# Autodesk Inventor assembly: DriveTrainPlate
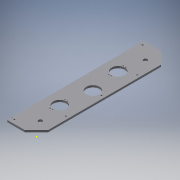
[picture p0: Inventor's stored thumbnail of the model, 180x180]
Saved by Autodesk Inventor 2017 (Build 210142000, 142)
## iProperties
Created: 2016-09-21
Part Number: DriveTrainPlate
Document SubType Name: Assembly
Designer: RoboticsUser
Author: RoboticsUser
## Documents named in this file (3)
- C:\Robotics\CAD\2016-17_CAD\DrainTrainPlate2.0.iam
- C:\Robotics\CAD\2016-17_CAD\DriveTrainPlate.ipt
- C:\Robotics\CAD\2016-17_CAD\Holefiller.ipt
## Components (4 placed, 2 different names)
1. DriveTrainPlate:1 — Mate:1, Flush:1, Mate:2, Flush:2, Mate:3, Flush:3
2. Holefiller:1 — Mate:1, Flush:1
3. Holefiller:2 — Mate:3, Flush:3
4. Holefiller:3 — Mate:2, Flush:2
## Relationships (6: Mate 3, Flush 3)
- Mate:1: DriveTrainPlate:1 ↔ Holefiller:1
- Flush:1: DriveTrainPlate:1 ↔ Holefiller:1
- Mate:2: DriveTrainPlate:1 ↔ Holefiller:3
- Flush:2: DriveTrainPlate:1 ↔ Holefiller:3
- Mate:3: DriveTrainPlate:1 ↔ Holefiller:2
- Flush:3: DriveTrainPlate:1 ↔ Holefiller:2
